# Autodesk Inventor assembly: 足全体_temp
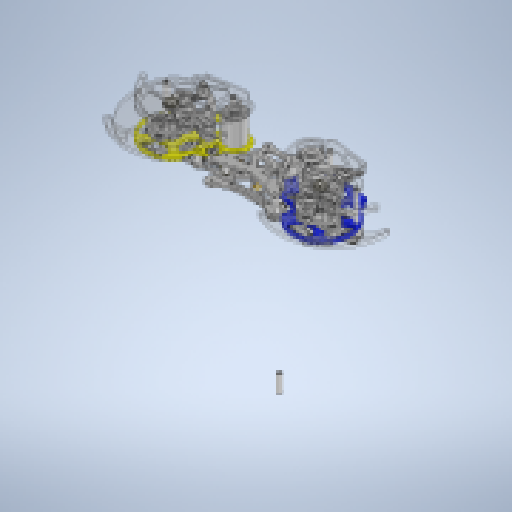
[picture p0: Inventor's stored thumbnail of the model, 512x512]
Saved by Autodesk Inventor 2023 (Build 270158000, 158)
## iProperties
Created: 2022-01-30
Part Number: 足全体_temp
Document SubType Name: Assembly
Designer: acps
Author: acps
## Documents named in this file (10)
- C:\Users\muzho\Documents\srdc\srdc_2\脚\足全体_temp.iam
- C:\Users\muzho\Documents\srdc\srdc_2\脚\足ユニット.iam
- C:\Users\muzho\Documents\srdc\srdc_2\スペーサ\l23.ipt
- C:\Users\muzho\Documents\srdc\srdc_2\タミヤダンパー1.iam
- C:\Users\muzho\Documents\srdc\srdc_2\スペーサ\l10.ipt
- C:\Users\muzho\Documents\srdc\srdc_2\脚\中間ユニット内_MIR1.ipt
- C:\Users\muzho\Documents\srdc\srdc_2\脚\中間ユニット外(shin).ipt
- C:\Users\muzho\Documents\srdc\srdc_2\脚\ミラー\足ユニット_MIR.iam
- C:\Users\muzho\Documents\srdc\srdc_2\脚\ミラー\l10_MIR.ipt
- C:\Users\muzho\Documents\srdc\srdc_2\脚\ミラー\l7_MIR.ipt
## Components (17 placed, 9 different names)
1. 足ユニット:1 [sub-assembly] — 挿入:23, メイト:10, 挿入:35
2. l23:1
3. l23:2
4. l23:3 — 挿入:33
5. l23:4 — メイト:10, 挿入:34
6. l23:5
7. l23:6 — 挿入:21
8. l23:7
9. l23:8 — メイト:5, 挿入:31, 挿入:32
10. タミヤダンパー1:1 [sub-assembly] — 挿入:24, メイト:11
11. l10:1 — 挿入:23, 挿入:24
12. 中間ユニット外(shin):1 — メイト:5, 挿入:21, メイト:9, 挿入:32, 挿入:33, 挿入:34, 挿入:35
13. 足ユニット_MIR:1 [sub-assembly] — 挿入:27
14. l10_MIR:1 — 挿入:27, メイト:8, 挿入:30
15. l7_MIR:1
16. タミヤダンパー1:2 [sub-assembly] — メイト:8, 挿入:30
17. 中間ユニット内_MIR1:2 — メイト:9, 挿入:31, メイト:11
## Relationships (15: Insert 10, Mate 5)
- メイト:5 [Mate]: l23:8 ↔ 中間ユニット外(shin):1
- 挿入:21 [Insert]: l23:6 ↔ 中間ユニット外(shin):1
- 挿入:23 [Insert]: 足ユニット:1 ↔ l10:1
- 挿入:24 [Insert]: タミヤダンパー1:1 ↔ l10:1
- 挿入:27 [Insert]: 足ユニット_MIR:1 ↔ l10_MIR:1
- メイト:8 [Mate]: l10_MIR:1 ↔ タミヤダンパー1:2
- 挿入:30 [Insert]: l10_MIR:1 ↔ タミヤダンパー1:2
- メイト:9 [Mate]: 中間ユニット外(shin):1 ↔ 中間ユニット内_MIR1:2
- 挿入:31 [Insert]: l23:8 ↔ 中間ユニット内_MIR1:2
- 挿入:32 [Insert]: l23:8 ↔ 中間ユニット外(shin):1
- 挿入:33 [Insert]: l23:3 ↔ 中間ユニット外(shin):1
- メイト:10 [Mate]: 足ユニット:1 ↔ l23:4
- 挿入:34 [Insert]: l23:4 ↔ 中間ユニット外(shin):1
- 挿入:35 [Insert] (0.5 mm): 足ユニット:1 ↔ 中間ユニット外(shin):1
- メイト:11 [Mate]: タミヤダンパー1:1 ↔ 中間ユニット内_MIR1:2
